# Autodesk Inventor assembly: Tower Assembly
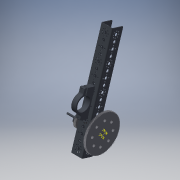
[picture p0: Inventor's stored thumbnail of the model, 180x180]
Saved by Autodesk Inventor 2016 (Build 200138000, 138)
## iProperties
Created: 2015-09-10
Part Number: Tower Assembly
Document SubType Name: Assembly
Designer: phiro
Author: phiro
## Documents named in this file (12)
- C:\Users\phiro\Documents\GitHub\phi_robotics\3d-models\FTC_Tetrix_KOP_Block_Party\Tim Bloot Designs\Tutorial Bot\Tower Assembly.iam
- C:\Users\phiro\Documents\GitHub\phi_robotics\3d-models\FTC_Tetrix_KOP_Block_Party\Tetrix_Kit_FTC\Autodesk Inventor Files\tetrix_gear-large.ipt
- C:\Users\phiro\Documents\GitHub\phi_robotics\3d-models\FTC_Tetrix_KOP_Block_Party\Tetrix_Kit_FTC\Autodesk Inventor Files\tetrix_axle_lock.iam
- C:\Users\phiro\Documents\GitHub\phi_robotics\3d-models\FTC_Tetrix_KOP_Block_Party\Tetrix_Kit_FTC\Autodesk Inventor Files\tetrix_screw.ipt
- C:\Users\phiro\Documents\GitHub\phi_robotics\3d-models\FTC_Tetrix_KOP_Block_Party\Tetrix_Kit_FTC\Autodesk Inventor Files\tetrix_axle.ipt
- C:\Users\phiro\Documents\GitHub\phi_robotics\3d-models\FTC_Tetrix_KOP_Block_Party\Tetrix_Kit_FTC\Autodesk Inventor Files\tetrix_c_channel-4.ipt
- C:\Users\phiro\Documents\GitHub\phi_robotics\3d-models\FTC_Tetrix_KOP_Block_Party\Tetrix_Kit_FTC\Autodesk Inventor Files\tetrix_bushing.ipt
- C:\Users\phiro\Documents\GitHub\phi_robotics\3d-models\FTC_Tetrix_KOP_Block_Party\Tetrix_Kit_FTC\Autodesk Inventor Files\tetrix_axle_spacer-big.ipt
- C:\Users\phiro\Documents\GitHub\phi_robotics\3d-models\FTC_Tetrix_KOP_Block_Party\Tetrix_Kit_FTC\Autodesk Inventor Files\tetrix_axle_spacer-small.ipt
- C:\Users\phiro\Documents\GitHub\phi_robotics\3d-models\FTC_Tetrix_KOP_Block_Party\Tetrix_Kit_FTC\Autodesk Inventor Files\tetrix_gear-small.ipt
- C:\Users\phiro\Documents\GitHub\phi_robotics\3d-models\FTC_Tetrix_KOP_Block_Party\Tetrix_Kit_FTC\Autodesk Inventor Files\tetrix_screw-buttonhead.ipt
- C:\Users\phiro\Documents\GitHub\phi_robotics\3d-models\FTC_Tetrix_KOP_Block_Party\Tetrix_Kit_FTC\Autodesk Inventor Files\tetrix_motor_mount-old.ipt
## Components (19 placed, 11 different names)
1. tetrix_gear-large:1 — Rigid:1, Rigid:2, Rigid:3, Rotational:1, Rotational:2, Rigid:4
2. tetrix_axle_lock:1 [sub-assembly] — Rigid:1, Rotational:12
3. tetrix_screw:1 — Rigid:3
4. tetrix_screw:2 — Rotational:1
5. tetrix_screw:3 — Rotational:2
6. tetrix_screw:4 — Rigid:2
7. tetrix_axle:1 — Rigid:4, Rigid:9
8. tetrix_c_channel-4:1 — Rotational:3, Rotational:4, Rigid:10
9. tetrix_bushing:1 — Rotational:4, Rotational:5
10. tetrix_bushing:2 — Rotational:3, Rotational:6
11. tetrix_axle_spacer-big:1 — Rotational:5, Rotational:12
12. tetrix_axle_spacer-small:1 — Rotational:6, Rotational:11
13. tetrix_gear-small:1 — Rigid:8, Rotational:7, Rotational:8, Rotational:9, Rotational:10, Rotational:11
14. tetrix_axle_lock:2 [sub-assembly] — Rigid:8, Rigid:9
15. tetrix_screw-buttonhead:1 — Rotational:10
16. tetrix_screw-buttonhead:2 — Rotational:9
17. tetrix_screw-buttonhead:3 — Rotational:7
18. tetrix_screw-buttonhead:4 — Rotational:8
19. tetrix_motor_mount-old:1 — Rigid:10
## Relationships (19: RevoluteJoint 12, WeldJoint 7)
- Rigid:1 [WeldJoint]: tetrix_gear-large:1 ↔ tetrix_axle_lock:1
- Rigid:2 [WeldJoint]: tetrix_gear-large:1 ↔ tetrix_screw:4
- Rigid:3 [WeldJoint]: tetrix_gear-large:1 ↔ tetrix_screw:1
- Rotational:1 [RevoluteJoint]: tetrix_gear-large:1 ↔ tetrix_screw:2
- Rotational:2 [RevoluteJoint]: tetrix_gear-large:1 ↔ tetrix_screw:3
- Rigid:4 [WeldJoint]: tetrix_gear-large:1 ↔ tetrix_axle:1
- Rotational:3 [RevoluteJoint]: tetrix_c_channel-4:1 ↔ tetrix_bushing:2
- Rotational:4 [RevoluteJoint]: tetrix_c_channel-4:1 ↔ tetrix_bushing:1
- Rotational:5 [RevoluteJoint]: tetrix_bushing:1 ↔ tetrix_axle_spacer-big:1
- Rotational:6 [RevoluteJoint]: tetrix_bushing:2 ↔ tetrix_axle_spacer-small:1
- Rigid:8 [WeldJoint]: tetrix_gear-small:1 ↔ tetrix_axle_lock:2
- Rotational:7 [RevoluteJoint]: tetrix_gear-small:1 ↔ tetrix_screw-buttonhead:3
- Rotational:8 [RevoluteJoint]: tetrix_gear-small:1 ↔ tetrix_screw-buttonhead:4
- Rotational:9 [RevoluteJoint]: tetrix_gear-small:1 ↔ tetrix_screw-buttonhead:2
- Rotational:10 [RevoluteJoint]: tetrix_gear-small:1 ↔ tetrix_screw-buttonhead:1
- Rotational:11 [RevoluteJoint]: tetrix_axle_spacer-small:1 ↔ tetrix_gear-small:1
- Rotational:12 [RevoluteJoint]: tetrix_axle_lock:1 ↔ tetrix_axle_spacer-big:1
- Rigid:9 [WeldJoint] (-26.25 mm): tetrix_axle:1 ↔ tetrix_axle_lock:2
- Rigid:10 [WeldJoint]: tetrix_c_channel-4:1 ↔ tetrix_motor_mount-old:1
